# Autodesk Inventor assembly: 리프트_회전부_ASSEMBLY
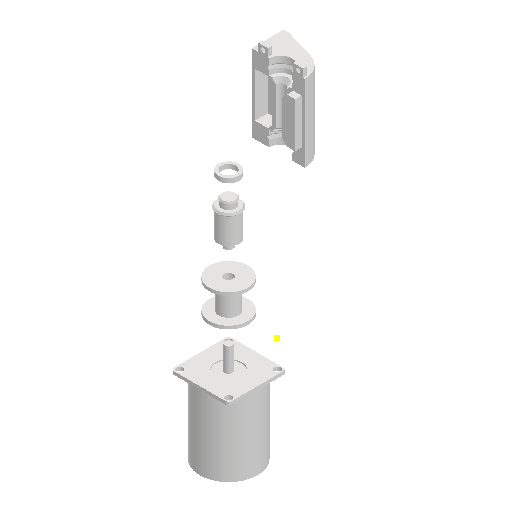
[picture p0: Inventor's stored thumbnail of the model, 512x512]
Saved by Autodesk Inventor 2027 (Build 310192000, 192)
## iProperties
Created: 2026-09-20
Part Number: 리프트_회전부_ASSEMBLY
Document SubType Name: Assembly
Designer: Kwon
Author: Kwon
## Documents named in this file (6)
- G:\다른 컴퓨터\내 컴퓨터\졸업작품\INVENTOR\리프트_회전부\리프트_회전부_ASSEMBLY.iam
- G:\다른 컴퓨터\내 컴퓨터\졸업작품\INVENTOR\리프트_회전부\모터.ipt
- G:\다른 컴퓨터\내 컴퓨터\졸업작품\INVENTOR\리프트_회전부\도르래.ipt
- G:\다른 컴퓨터\내 컴퓨터\졸업작품\INVENTOR\리프트_회전부\안쪽_베어링 고정부.ipt
- G:\다른 컴퓨터\내 컴퓨터\졸업작품\INVENTOR\리프트_회전부\베어링.ipt
- G:\다른 컴퓨터\내 컴퓨터\졸업작품\INVENTOR\리프트_회전부\바깥쪽_베어링 고정부_split1.ipt
## Components (5 placed, 5 different names)
1. 모터:1 — Insert:1
2. 도르래:1 — Insert:1, Insert:2
3. 안쪽_베어링 고정부:1 — Insert:2, Insert:3
4. 베어링:1 — Insert:3, Mate:1
5. 바깥쪽_베어링 고정부_split1:1 — Mate:1
## Relationships (4: Insert 3, Mate 1)
- Insert:1 (40 mm): 모터:1 ↔ 도르래:1
- Insert:2 (40 mm): 도르래:1 ↔ 안쪽_베어링 고정부:1
- Insert:3 (40 mm): 안쪽_베어링 고정부:1 ↔ 베어링:1
- Mate:1 (80 mm): 베어링:1 ↔ 바깥쪽_베어링 고정부_split1:1
